# Autodesk Inventor assembly: KPA4C
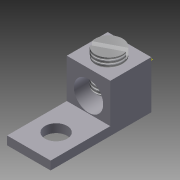
[picture p0: Inventor's stored thumbnail of the model, 180x180]
Saved by Autodesk Inventor 2013 (Build 170138000, 138)
## iProperties
Shininess: 64.0
Angle Display Precision: 2
Document Length Units: 11272
Document Angle Units: 11279
Document Time Units: 11290
Document Mass Units: 11286
Document Length Units Precision: 3
Document Angle Units Precision: 2
Category: Electrical
Company: Autodesk Inc.
Created: 2008-12-14
Part Number: KPA4C
Catalog Web Link: http://portal.fciconnect.com/portal/page/portal/FcicntPublic/ComergentConnect?appname=catDisplayStyle$domProductQueryName=kpa4c*$OP=search
Description: Terminal lug, 6-14ga solderless lug
Vendor: FCI Burndy
Document SubType Name: Assembly
Designer: Autodesk Inc.
Density: 0.0
Volumn: 0.0
Area: 0.0
PropertySet Name: Model Information
Control State: 0
Master: False
Checked Out: False
Author: Autodesk Inc.
## Documents named in this file (3)
- \\lmss\STUDENTS\Robotics\CAD Files\COTS Parts\vkop\All-Electrical\Terminal Lug _Burndy_KPA4C.iam
- \\lmss\STUDENTS\Robotics\CAD Files\COTS Parts\vkop\All-Electrical\Terminal Battery.ipt
- \\lmss\STUDENTS\Robotics\CAD Files\COTS Parts\vkop\All-Electrical\Terminal Screw.ipt
## Components (2 placed, 2 different names)
1. Terminal Battery:1 — Mate:1, Flush:1
2. Terminal Screw:1 — Mate:1, Flush:1
## Relationships (2: Mate 1, Flush 1)
- Mate:1: Terminal Battery:1 ↔ Terminal Screw:1
- Flush:1 (-2.54 mm): Terminal Battery:1 ↔ Terminal Screw:1
